# Autodesk Inventor assembly: 217-3433-Fully Constrained
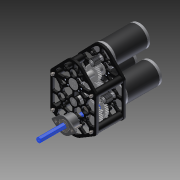
[picture p0: Inventor's stored thumbnail of the model, 180x180]
Saved by Autodesk Inventor 2014 SP1 (Build 180222100, 222)
## iProperties
Created: 2014-01-04
Part Number: 217-3433-Fully Constrained
Document SubType Name: Assembly
Designer: Moses
Mass: 6071.56 g
Surface Area: 3557.48 cm^2
Volume: 1472.05 cm^3
Density: 4.12457 g/cm^3
Title: 217-3433-STEP.STEP
Description: STEP AP214
Creation Date: 2013-12-10
Sending System: SolidWorks 2013
Preprocessor: SwSTEP 2.0
Author: Moses
## Documents named in this file (44)
- C:\Users\Arpan\Documents\GitHub\2014buildCAD\chassisdrivetrain\gearbot\217-3433 (3 CIM Gearbox - WC)\217-3433-Fully Constrained.iam
- C:\Users\Arpan\Documents\GitHub\2014buildCAD\chassisdrivetrain\gearbot\217-3433 (3 CIM Gearbox - WC)\217-2428-027 Rev1_97414A630.ipt
- C:\Users\Arpan\Documents\GitHub\2014buildCAD\chassisdrivetrain\gearbot\217-3433 (3 CIM Gearbox - WC)\217-3423-005 Rev1.ipt
- C:\Users\Arpan\Documents\GitHub\2014buildCAD\chassisdrivetrain\gearbot\217-3433 (3 CIM Gearbox - WC)\217-3195-200 Rev1.iam
- C:\Users\Arpan\Documents\GitHub\2014buildCAD\chassisdrivetrain\gearbot\217-3433 (3 CIM Gearbox - WC)\217-3489.ipt
- C:\Users\Arpan\Documents\GitHub\2014buildCAD\chassisdrivetrain\gearbot\217-3433 (3 CIM Gearbox - WC)\217-3423-006 Rev1.ipt
- C:\Users\Arpan\Documents\GitHub\2014buildCAD\chassisdrivetrain\gearbot\217-3433 (3 CIM Gearbox - WC)\217-3423-008 Rev1.ipt
- C:\Users\Arpan\Documents\GitHub\2014buildCAD\chassisdrivetrain\gearbot\217-3433 (3 CIM Gearbox - WC)\217-3423-009 Rev1.ipt
- C:\Users\Arpan\Documents\GitHub\2014buildCAD\chassisdrivetrain\gearbot\217-3433 (3 CIM Gearbox - WC)\217-2778-001 Rev2_NCQ8A075-050M.iam
- C:\Users\Arpan\Documents\GitHub\2014buildCAD\chassisdrivetrain\gearbot\217-3433 (3 CIM Gearbox - WC)\217-2731.ipt
- C:\Users\Arpan\Documents\GitHub\2014buildCAD\chassisdrivetrain\gearbot\217-3433 (3 CIM Gearbox - WC)\217-2733.ipt
- C:\Users\Arpan\Documents\GitHub\2014buildCAD\chassisdrivetrain\gearbot\217-3433 (3 CIM Gearbox - WC)\217-2734.ipt
- C:\Users\Arpan\Documents\GitHub\2014buildCAD\chassisdrivetrain\gearbot\217-3433 (3 CIM Gearbox - WC)\217-2743.ipt
- C:\Users\Arpan\Documents\GitHub\2014buildCAD\chassisdrivetrain\gearbot\217-3433 (3 CIM Gearbox - WC)\217-2614-002_98430A132.ipt
- C:\Users\Arpan\Documents\GitHub\2014buildCAD\chassisdrivetrain\gearbot\217-3433 (3 CIM Gearbox - WC)\217-3421-007 Rev1.ipt
- C:\Users\Arpan\Documents\GitHub\2014buildCAD\chassisdrivetrain\gearbot\217-3433 (3 CIM Gearbox - WC)\217-3421-009 Rev1.ipt
- C:\Users\Arpan\Documents\GitHub\2014buildCAD\chassisdrivetrain\gearbot\217-3433 (3 CIM Gearbox - WC)\217-3421-010 Rev1.ipt
- C:\Users\Arpan\Documents\GitHub\2014buildCAD\chassisdrivetrain\gearbot\217-3433 (3 CIM Gearbox - WC)\217-3421-011 Rev2_97633A200.ipt
- C:\Users\Arpan\Documents\GitHub\2014buildCAD\chassisdrivetrain\gearbot\217-3433 (3 CIM Gearbox - WC)\217-3422-007 Rev1.ipt
- C:\Users\Arpan\Documents\GitHub\2014buildCAD\chassisdrivetrain\gearbot\217-3433 (3 CIM Gearbox - WC)\217-3423-014 Rev1.ipt
- C:\Users\Arpan\Documents\GitHub\2014buildCAD\chassisdrivetrain\gearbot\217-3433 (3 CIM Gearbox - WC)\217-3423-016 Rev1.ipt
- C:\Users\Arpan\Documents\GitHub\2014buildCAD\chassisdrivetrain\gearbot\217-3433 (3 CIM Gearbox - WC)\217-3424-003 Rev1.ipt
- C:\Users\Arpan\Documents\GitHub\2014buildCAD\chassisdrivetrain\gearbot\217-3433 (3 CIM Gearbox - WC)\217-2761-001 rev1.ipt
- C:\Users\Arpan\Documents\GitHub\2014buildCAD\chassisdrivetrain\gearbot\217-3433 (3 CIM Gearbox - WC)\217-3210-001 Rev1_30t.ipt
- C:\Users\Arpan\Documents\GitHub\2014buildCAD\chassisdrivetrain\gearbot\217-3433 (3 CIM Gearbox - WC)\217-3215-001 Rev1_42t.ipt
- C:\Users\Arpan\Documents\GitHub\2014buildCAD\chassisdrivetrain\gearbot\217-3433 (3 CIM Gearbox - WC)\217-3414-001 Rev1_14t Steel Pinion.ipt
- C:\Users\Arpan\Documents\GitHub\2014buildCAD\chassisdrivetrain\gearbot\217-3433 (3 CIM Gearbox - WC)\217-3418-001 Rev2_44t.ipt
- C:\Users\Arpan\Documents\GitHub\2014buildCAD\chassisdrivetrain\gearbot\217-3433 (3 CIM Gearbox - WC)\217-3420-001 Rev2_60t.ipt
- C:\Users\Arpan\Documents\GitHub\2014buildCAD\chassisdrivetrain\gearbot\217-3433 (3 CIM Gearbox - WC)\217-3100-001_14t.ipt
- C:\Users\Arpan\Documents\GitHub\2014buildCAD\chassisdrivetrain\gearbot\217-3433 (3 CIM Gearbox - WC)\217-2705-001_30t.ipt
- C:\Users\Arpan\Documents\GitHub\2014buildCAD\chassisdrivetrain\gearbot\217-3433 (3 CIM Gearbox - WC)\217-2000.ipt
- C:\Users\Arpan\Documents\GitHub\2014buildCAD\chassisdrivetrain\gearbot\217-3433 (3 CIM Gearbox - WC)\217-3433-001 Rev1_Default_As Machined_.ipt
- C:\Users\Arpan\Documents\GitHub\2014buildCAD\chassisdrivetrain\gearbot\217-3433 (3 CIM Gearbox - WC)\217-3423-003 Rev1.ipt
- C:\Users\Arpan\Documents\GitHub\2014buildCAD\chassisdrivetrain\gearbot\217-3433 (3 CIM Gearbox - WC)\217-3424-005 Rev1.ipt
- C:\Users\Arpan\Documents\GitHub\2014buildCAD\chassisdrivetrain\gearbot\217-3433 (3 CIM Gearbox - WC)\217-3433-003 Rev1.ipt
- C:\Users\Arpan\Documents\GitHub\2014buildCAD\chassisdrivetrain\gearbot\217-3433 (3 CIM Gearbox - WC)\217-3256-001 Rev1.ipt
- C:\Users\Arpan\Documents\GitHub\2014buildCAD\chassisdrivetrain\gearbot\217-3433 (3 CIM Gearbox - WC)\217-3261-001 Rev1.ipt
- C:\Users\Arpan\Documents\GitHub\2014buildCAD\chassisdrivetrain\gearbot\217-3433 (3 CIM Gearbox - WC)\217-3423-004 Rev1.ipt
- C:\Users\Arpan\Documents\GitHub\2014buildCAD\chassisdrivetrain\gearbot\217-3433 (3 CIM Gearbox - WC)\217-3424-002 Rev1.ipt
- C:\Users\Arpan\Documents\GitHub\2014buildCAD\chassisdrivetrain\gearbot\217-3433 (3 CIM Gearbox - WC)\217-3422-004 Rev2.ipt
- C:\Users\Arpan\Documents\GitHub\2014buildCAD\chassisdrivetrain\gearbot\217-3433 (3 CIM Gearbox - WC)\217-3257-001 Rev1.ipt
- C:\Users\Arpan\Documents\GitHub\2014buildCAD\chassisdrivetrain\gearbot\217-3433 (3 CIM Gearbox - WC)\217-3263-001 Rev1.ipt
- C:\Users\Arpan\Documents\GitHub\2014buildCAD\chassisdrivetrain\gearbot\217-3433 (3 CIM Gearbox - WC)\217-3259-001 Rev1.ipt
- C:\Users\Arpan\Documents\GitHub\2014buildCAD\chassisdrivetrain\gearbot\217-3433 (3 CIM Gearbox - WC)\217-2758-001 Rev1.ipt
## Components (78 placed, 78 different names)
1. 217-2428-027 Rev1_97414A630_1 — Insert:47, Mate:62, Rotation:10
2. 217-3423-005 Rev1_2 — Insert:32, Insert:33, Insert:34, Insert:35, Insert:36, Mate:61
3. 217-3195-200 Rev1_3 [sub-assembly] — Flush:4, Mate:60, Mate:61, Rotation:9, Angle:13
4. 217-3489_4 — Insert:47, Mate:64
5. 217-3423-006 Rev1_5 — Insert:31, Insert:32
6. 217-3423-006 Rev1_6 — Insert:30, Insert:33
7. 217-3423-008 Rev1_7 — Mate:29, Mate:42, Flush:4, Mate:60, Mate:62, Mate:64
8. 217-3423-009 Rev1_8 — Mate:34, Insert:28, Rotation:2
9. 217-2778-001 Rev2_NCQ8A075-050M_9 [sub-assembly] — Insert:36, Angle:6, Angle:13
10. 217-2731_10 — Insert:22, Mate:24, Mate:29, Mate:43, Mate:45
11. 217-2733_11 — Insert:40, Insert:45
12. 217-2733_12 — Insert:15, Insert:38
13. 217-2734_13 — Insert:13, Angle:1, Flush:3, Insert:48
14. 217-2734_14 — Insert:27, Angle:2, Mate:35, Mate:36
15. 217-2743_15 — Mate:39, Mate:40
16. 217-2731_16 — Insert:12, Insert:37
17. 217-2731_17 — Insert:41, Insert:46
18. 217-2614-002_98430A132_18 — Mate:27, Mate:47, Rotation:13
19. 217-2614-002_98430A132_19 — Mate:28, Mate:48, Rotation:16
20. 217-2614-002_98430A132_20 — Mate:51, Mate:54, Rotation:12
21. 217-2614-002_98430A132_21 — Mate:52, Mate:53, Rotation:15
22. 217-2614-002_98430A132_22 — Mate:25, Mate:50, Rotation:11
23. 217-2614-002_98430A132_23 — Mate:26, Mate:49, Rotation:14
24. 217-3421-007 Rev1_24 — Insert:34
25. 217-3421-007 Rev1_25 — Insert:35
26. 217-3421-009 Rev1_26 — Insert:19
27. 217-3421-009 Rev1_27 — Insert:17
28. 217-3421-009 Rev1_28 — Insert:18
29. 217-3421-009 Rev1_29 — Insert:21
30. 217-3421-009 Rev1_30 — Insert:20
31. 217-3421-009 Rev1_31 — Insert:16
32. 217-3421-010 Rev1_32 — Insert:26
33. 217-3421-010 Rev1_33 — Insert:25
34. 217-3421-010 Rev1_34 — Insert:23
35. 217-3421-010 Rev1_35 — Insert:24
36. 217-3421-011 Rev2_97633A200_36 — Insert:29, Rotation:4
37. 217-3422-007 Rev1_37 — Flush:1, Mate:5, Mate:7
38. 217-3422-007 Rev1_38 — Flush:2, Mate:6, Mate:8
39. 217-3423-014 Rev1_39 — Insert:28, Mate:42
40. 217-3423-016 Rev1_40 — Mate:45, Mate:46
41. 217-3423-016 Rev1_41 — Mate:43, Mate:44
42. 217-3423-016 Rev1_42 — Mate:23, Mate:24
43. 217-3424-003 Rev1_43 — Insert:59
44. 217-3424-003 Rev1_44 — Insert:60
45. 217-3424-003 Rev1_45 — Insert:58
46. 217-3424-003 Rev1_46 — Insert:57
47. 217-2761-001 rev1_47 — Mate:20, Mate:21, Mate:22
48. 217-2761-001 rev1_48 — Mate:4, Mate:13, Mate:14
49. 217-2761-001 rev1_49 — Mate:15, Mate:16, Mate:18
50. 217-3210-001 Rev1_30t_50 — Insert:44, Angle:11, Insert:45, Rotation:18
51. 217-3215-001 Rev1_42t_51 — Insert:43, Mate:59, Angle:10, Insert:44, Rotation:6, Rotation:7, Rotation:8
52. 217-3414-001 Rev1_14t Steel Pinion_52 — Mate:3, Mate:11, Mate:52, Mate:54, Rotation:7, Rotation:12, Rotation:15
53. 217-3414-001 Rev1_14t Steel Pinion_53 — Mate:2, Mate:10, Mate:47, Mate:48, Rotation:8, Rotation:13, Rotation:16
54. 217-3414-001 Rev1_14t Steel Pinion_54 — Mate:1, Mate:9, Mate:49, Mate:50, Rotation:5, Rotation:11, Rotation:14
55. 217-3418-001 Rev2_44t_55 — Mate:37, Fast Rotation Ratio:3, Mate:40, Mate:41, Rotation:18
56. 217-3420-001 Rev2_60t_56 — Insert:27, Slow Rotation Ratio:1, Mate:41, Rotation:17
57. 217-3100-001_14t_57 — Angle:7, Insert:39, Rotation:17
58. 217-2705-001_30t_58 — Angle:8, Insert:42, Rotation:5, Rotation:6
59. 217-2000_59 — Insert:2, Mate:2, Mate:10, Mate:19, Mate:20, Mate:21, Mate:22, Mate:27, Mate:28
60. 217-2000_60 — Insert:3, Mate:3, Mate:4, Mate:11, Mate:12, Mate:13, Mate:14, Mate:51, Mate:53
61. 217-2000_61 — Insert:1, Mate:1, Mate:9, Mate:15, Mate:16, Mate:17, Mate:18, Mate:25, Mate:26
62. 217-3433-001 Rev1_Default<As Machined>_62 — Insert:1, Insert:2, Insert:3, Insert:4, Insert:7, Insert:8, Insert:11, Insert:16, Insert:17, Insert:18, Insert:19, Insert:20, Insert:21, Mate:12, Mate:17, Mate:19, Insert:22, Mate:23, Insert:23, Insert:24, Insert:25, Insert:26, Insert:30, Insert:31, Angle:6, Mate:44, Mate:46, Insert:40, Insert:41
63. 217-3433-001 Rev1_Default<As Machined>_63 — Insert:5, Insert:6, Insert:9, Insert:10, Insert:12, Mate:5, Mate:6, Insert:14, Insert:15, Mate:30, Mate:31, Mate:32, Mate:33, Mate:34, Mate:35, Mate:37, Mate:38, Mate:39, Insert:58, Insert:57, Insert:60, Insert:59
64. 217-3423-003 Rev1_64 — Angle:1, Slow Rotation Ratio:1, Angle:2, Rotation:2, Mate:36, Fast Rotation Ratio:3, Mate:38, Flush:3, Angle:3, Angle:4, Angle:5, Insert:29, Rotation:4, Rotation:9, Rotation:10
65. 217-3424-005 Rev1_65 — Insert:38, Angle:7, Insert:39, Angle:9, Mate:59, Angle:10, Angle:11
66. 217-3433-003 Rev1_66 — Insert:37, Angle:8, Insert:42, Angle:12
67. 217-3256-001 Rev1_67 — Insert:43, Angle:9
68. 217-3261-001 Rev1_68 — Insert:46, Angle:12
69. 217-3423-004 Rev1_69
70. 217-3424-002 Rev1_70 — Insert:6, Insert:7
71. 217-3424-002 Rev1_71 — Insert:10, Insert:11
72. 217-3424-002 Rev1_72 — Insert:4, Insert:5
73. 217-3424-002 Rev1_73 — Insert:8, Insert:9
74. 217-3422-004 Rev2_74 — Insert:13, Flush:1, Flush:2, Mate:7, Mate:8, Insert:14
75. 217-3257-001 Rev1_75 — Mate:33, Angle:3
76. 217-3263-001 Rev1_76 — Mate:30, Insert:48, Insert:49
77. 217-3259-001 Rev1_77 — Mate:31, Angle:5, Mate:63, Insert:49
78. 217-2758-001 Rev1_78 — Mate:32, Angle:4, Mate:63
## Relationships (148: Mate 60, Insert 53, RelateRotation 18, Angle 13, Flush 4)
- Insert:1: 217-2000_61 ↔ 217-3433-001 Rev1_Default<As Machined>_62
- Insert:2: 217-2000_59 ↔ 217-3433-001 Rev1_Default<As Machined>_62
- Insert:3: 217-2000_60 ↔ 217-3433-001 Rev1_Default<As Machined>_62
- Mate:1 (10.2113 mm): 217-3414-001 Rev1_14t Steel Pinion_54 ↔ 217-2000_61
- Mate:2 (10.2113 mm): 217-3414-001 Rev1_14t Steel Pinion_53 ↔ 217-2000_59
- Mate:3 (10.2113 mm): 217-3414-001 Rev1_14t Steel Pinion_52 ↔ 217-2000_60
- Mate:4: 217-2761-001 rev1_48 ↔ 217-2000_60
- Insert:4: 217-3433-001 Rev1_Default<As Machined>_62 ↔ 217-3424-002 Rev1_72
- Insert:5: 217-3433-001 Rev1_Default<As Machined>_63 ↔ 217-3424-002 Rev1_72
- Insert:6: 217-3433-001 Rev1_Default<As Machined>_63 ↔ 217-3424-002 Rev1_70
- Insert:7: 217-3433-001 Rev1_Default<As Machined>_62 ↔ 217-3424-002 Rev1_70
- Insert:8: 217-3433-001 Rev1_Default<As Machined>_62 ↔ 217-3424-002 Rev1_73
- Insert:9: 217-3433-001 Rev1_Default<As Machined>_63 ↔ 217-3424-002 Rev1_73
- Insert:10: 217-3433-001 Rev1_Default<As Machined>_63 ↔ 217-3424-002 Rev1_71
- Insert:11: 217-3433-001 Rev1_Default<As Machined>_62 ↔ 217-3424-002 Rev1_71
- Insert:12: 217-2731_16 ↔ 217-3433-001 Rev1_Default<As Machined>_63
- Insert:13: 217-2734_13 ↔ 217-3422-004 Rev2_74
- Flush:1: 217-3422-007 Rev1_37 ↔ 217-3422-004 Rev2_74
- Flush:2: 217-3422-007 Rev1_38 ↔ 217-3422-004 Rev2_74
- Mate:5: 217-3422-007 Rev1_37 ↔ 217-3433-001 Rev1_Default<As Machined>_63
- Mate:6: 217-3422-007 Rev1_38 ↔ 217-3433-001 Rev1_Default<As Machined>_63
- Mate:7: 217-3422-007 Rev1_37 ↔ 217-3422-004 Rev2_74
- Mate:8: 217-3422-007 Rev1_38 ↔ 217-3422-004 Rev2_74
- Insert:14: 217-3433-001 Rev1_Default<As Machined>_63 ↔ 217-3422-004 Rev2_74
- Insert:15: 217-2733_12 ↔ 217-3433-001 Rev1_Default<As Machined>_63
- Insert:16: 217-3421-009 Rev1_31 ↔ 217-3433-001 Rev1_Default<As Machined>_62
- Insert:17: 217-3421-009 Rev1_27 ↔ 217-3433-001 Rev1_Default<As Machined>_62
- Insert:18: 217-3421-009 Rev1_28 ↔ 217-3433-001 Rev1_Default<As Machined>_62
- Insert:19: 217-3421-009 Rev1_26 ↔ 217-3433-001 Rev1_Default<As Machined>_62
- Mate:9: 217-3414-001 Rev1_14t Steel Pinion_54 ↔ 217-2000_61
- Mate:10: 217-3414-001 Rev1_14t Steel Pinion_53 ↔ 217-2000_59
- Mate:11: 217-3414-001 Rev1_14t Steel Pinion_52 ↔ 217-2000_60
- Insert:20: 217-3421-009 Rev1_30 ↔ 217-3433-001 Rev1_Default<As Machined>_62
- Insert:21: 217-3421-009 Rev1_29 ↔ 217-3433-001 Rev1_Default<As Machined>_62
- Mate:12: 217-2000_60 ↔ 217-3433-001 Rev1_Default<As Machined>_62
- Mate:13: 217-2761-001 rev1_48 ↔ 217-2000_60
- Mate:14: 217-2761-001 rev1_48 ↔ 217-2000_60
- Mate:15: 217-2761-001 rev1_49 ↔ 217-2000_61
- Mate:16: 217-2761-001 rev1_49 ↔ 217-2000_61
- Mate:17: 217-2000_61 ↔ 217-3433-001 Rev1_Default<As Machined>_62
- Mate:18: 217-2761-001 rev1_49 ↔ 217-2000_61
- Mate:19: 217-2000_59 ↔ 217-3433-001 Rev1_Default<As Machined>_62
- Mate:20: 217-2761-001 rev1_47 ↔ 217-2000_59
- Mate:21: 217-2761-001 rev1_47 ↔ 217-2000_59
- Mate:22: 217-2761-001 rev1_47 ↔ 217-2000_59
- Insert:22: 217-2731_10 ↔ 217-3433-001 Rev1_Default<As Machined>_62
- Mate:23: 217-3423-016 Rev1_42 ↔ 217-3433-001 Rev1_Default<As Machined>_62
- Mate:24: 217-2731_10 ↔ 217-3423-016 Rev1_42
- Mate:25: 217-2614-002_98430A132_22 ↔ 217-2000_61
- Mate:26: 217-2614-002_98430A132_23 ↔ 217-2000_61
- Mate:27: 217-2614-002_98430A132_18 ↔ 217-2000_59
- Mate:28: 217-2614-002_98430A132_19 ↔ 217-2000_59
- Mate:29: 217-3423-008 Rev1_7 ↔ 217-2731_10
- Angle:1 (0 deg): 217-2734_13 ↔ 217-3423-003 Rev1_64
- Insert:23: 217-3421-010 Rev1_34 ↔ 217-3433-001 Rev1_Default<As Machined>_62
- Insert:24: 217-3421-010 Rev1_35 ↔ 217-3433-001 Rev1_Default<As Machined>_62
- Insert:25: 217-3421-010 Rev1_33 ↔ 217-3433-001 Rev1_Default<As Machined>_62
- Insert:26: 217-3421-010 Rev1_32 ↔ 217-3433-001 Rev1_Default<As Machined>_62
- Mate:30: 217-3433-001 Rev1_Default<As Machined>_63 ↔ 217-3263-001 Rev1_76
- Mate:31: 217-3433-001 Rev1_Default<As Machined>_63 ↔ 217-3259-001 Rev1_77
- Mate:32: 217-3433-001 Rev1_Default<As Machined>_63 ↔ 217-2758-001 Rev1_78
- Mate:33: 217-3433-001 Rev1_Default<As Machined>_63 ↔ 217-3257-001 Rev1_75
- Insert:27: 217-2734_14 ↔ 217-3420-001 Rev2_60t_56
- Mate:34: 217-3423-009 Rev1_8 ↔ 217-3433-001 Rev1_Default<As Machined>_63
- Insert:28: 217-3423-009 Rev1_8 ↔ 217-3423-014 Rev1_39
- Slow Rotation Ratio:1 [RelateRotation] (1 ul): 217-3420-001 Rev2_60t_56 ↔ 217-3423-003 Rev1_64
- Angle:2 (0 deg): 217-2734_14 ↔ 217-3423-003 Rev1_64
- Rotation:2 [RelateRotation] (1 ul): 217-3423-009 Rev1_8 ↔ 217-3423-003 Rev1_64
- Mate:35: 217-2734_14 ↔ 217-3433-001 Rev1_Default<As Machined>_63
- Mate:36: 217-2734_14 ↔ 217-3423-003 Rev1_64
- Mate:37: 217-3418-001 Rev2_44t_55 ↔ 217-3433-001 Rev1_Default<As Machined>_63
- Fast Rotation Ratio:3 [RelateRotation] (1 ul): 217-3418-001 Rev2_44t_55 ↔ 217-3423-003 Rev1_64
- Mate:38: 217-3433-001 Rev1_Default<As Machined>_63 ↔ 217-3423-003 Rev1_64
- Flush:3 (74.8347 mm): 217-2734_13 ↔ 217-3423-003 Rev1_64
- Angle:3 (0 deg): 217-3423-003 Rev1_64 ↔ 217-3257-001 Rev1_75
- Angle:4 (0 deg): 217-3423-003 Rev1_64 ↔ 217-2758-001 Rev1_78
- Angle:5 (0 deg): 217-3423-003 Rev1_64 ↔ 217-3259-001 Rev1_77
- Mate:39: 217-2743_15 ↔ 217-3433-001 Rev1_Default<As Machined>_63
- Mate:40: 217-2743_15 ↔ 217-3418-001 Rev2_44t_55
- Mate:41 (18.1613 mm): 217-3418-001 Rev2_44t_55 ↔ 217-3420-001 Rev2_60t_56
- Mate:42: 217-3423-008 Rev1_7 ↔ 217-3423-014 Rev1_39
- Insert:29: 217-3421-011 Rev2_97633A200_36 ↔ 217-3423-003 Rev1_64
- Rotation:4 [RelateRotation] (1 ul): 217-3421-011 Rev2_97633A200_36 ↔ 217-3423-003 Rev1_64
- Insert:30: 217-3423-006 Rev1_6 ↔ 217-3433-001 Rev1_Default<As Machined>_62
- Insert:31: 217-3423-006 Rev1_5 ↔ 217-3433-001 Rev1_Default<As Machined>_62
- Insert:32: 217-3423-005 Rev1_2 ↔ 217-3423-006 Rev1_5
- Insert:33: 217-3423-005 Rev1_2 ↔ 217-3423-006 Rev1_6
- Insert:34: 217-3423-005 Rev1_2 ↔ 217-3421-007 Rev1_24
- Insert:35: 217-3423-005 Rev1_2 ↔ 217-3421-007 Rev1_25
- Flush:4: 217-3195-200 Rev1_3 ↔ 217-3423-008 Rev1_7
- Insert:36: 217-3423-005 Rev1_2 ↔ 217-2778-001 Rev2_NCQ8A075-050M_9
- Angle:6 (0 deg): 217-2778-001 Rev2_NCQ8A075-050M_9 ↔ 217-3433-001 Rev1_Default<As Machined>_62
- Mate:43: 217-2731_10 ↔ 217-3423-016 Rev1_41
- Mate:44: 217-3423-016 Rev1_41 ↔ 217-3433-001 Rev1_Default<As Machined>_62
- Mate:45: 217-2731_10 ↔ 217-3423-016 Rev1_40
- Mate:46: 217-3423-016 Rev1_40 ↔ 217-3433-001 Rev1_Default<As Machined>_62
- Insert:37: 217-2731_16 ↔ 217-3433-003 Rev1_66
- Insert:38: 217-2733_12 ↔ 217-3424-005 Rev1_65
- Mate:47: 217-2614-002_98430A132_18 ↔ 217-3414-001 Rev1_14t Steel Pinion_53
- Mate:48: 217-2614-002_98430A132_19 ↔ 217-3414-001 Rev1_14t Steel Pinion_53
- Mate:49: 217-2614-002_98430A132_23 ↔ 217-3414-001 Rev1_14t Steel Pinion_54
- Mate:50: 217-2614-002_98430A132_22 ↔ 217-3414-001 Rev1_14t Steel Pinion_54
- Mate:51: 217-2614-002_98430A132_20 ↔ 217-2000_60
- Mate:52: 217-2614-002_98430A132_21 ↔ 217-3414-001 Rev1_14t Steel Pinion_52
- Mate:53: 217-2614-002_98430A132_21 ↔ 217-2000_60
- Mate:54: 217-2614-002_98430A132_20 ↔ 217-3414-001 Rev1_14t Steel Pinion_52
- Insert:58 (3.175 mm): 217-3424-003 Rev1_45 ↔ 217-3433-001 Rev1_Default<As Machined>_63
- Insert:57 (3.175 mm): 217-3424-003 Rev1_46 ↔ 217-3433-001 Rev1_Default<As Machined>_63
- Insert:60 (3.175 mm): 217-3424-003 Rev1_44 ↔ 217-3433-001 Rev1_Default<As Machined>_63
- Insert:59 (3.175 mm): 217-3424-003 Rev1_43 ↔ 217-3433-001 Rev1_Default<As Machined>_63
- Angle:7 (0 deg): 217-3100-001_14t_57 ↔ 217-3424-005 Rev1_65
- Insert:39: 217-3100-001_14t_57 ↔ 217-3424-005 Rev1_65
- Insert:40: 217-2733_11 ↔ 217-3433-001 Rev1_Default<As Machined>_62
- Insert:41: 217-2731_17 ↔ 217-3433-001 Rev1_Default<As Machined>_62
- Angle:8 (0 deg): 217-2705-001_30t_58 ↔ 217-3433-003 Rev1_66
- Insert:42: 217-2705-001_30t_58 ↔ 217-3433-003 Rev1_66
- Insert:43: 217-3215-001 Rev1_42t_51 ↔ 217-3256-001 Rev1_67
- Angle:9 (0 deg): 217-3424-005 Rev1_65 ↔ 217-3256-001 Rev1_67
- Mate:59: 217-3215-001 Rev1_42t_51 ↔ 217-3424-005 Rev1_65
- Angle:10 (0 deg): 217-3215-001 Rev1_42t_51 ↔ 217-3424-005 Rev1_65
- Insert:44: 217-3210-001 Rev1_30t_50 ↔ 217-3215-001 Rev1_42t_51
- Angle:11 (0 deg): 217-3210-001 Rev1_30t_50 ↔ 217-3424-005 Rev1_65
- Insert:45: 217-2733_11 ↔ 217-3210-001 Rev1_30t_50
- Insert:46: 217-2731_17 ↔ 217-3261-001 Rev1_68
- Angle:12 (0 deg): 217-3433-003 Rev1_66 ↔ 217-3261-001 Rev1_68
- Rotation:5 [RelateRotation] (2.1429 ul): 217-3414-001 Rev1_14t Steel Pinion_54 ↔ 217-2705-001_30t_58
- Rotation:6 [RelateRotation] (0.7143 ul): 217-3215-001 Rev1_42t_51 ↔ 217-2705-001_30t_58
- Rotation:7 [RelateRotation] (3 ul): 217-3215-001 Rev1_42t_51 ↔ 217-3414-001 Rev1_14t Steel Pinion_52
- Rotation:8 [RelateRotation] (3 ul): 217-3215-001 Rev1_42t_51 ↔ 217-3414-001 Rev1_14t Steel Pinion_53
- Mate:60: 217-3195-200 Rev1_3 ↔ 217-3423-008 Rev1_7
- Mate:61 (4.7711 mm): 217-3423-005 Rev1_2 ↔ 217-3195-200 Rev1_3
- Rotation:9 [RelateRotation] (1 ul): 217-3195-200 Rev1_3 ↔ 217-3423-003 Rev1_64
- Insert:47: 217-2428-027 Rev1_97414A630_1 ↔ 217-3489_4
- Mate:62 (0.0908 mm): 217-2428-027 Rev1_97414A630_1 ↔ 217-3423-008 Rev1_7
- Angle:13 (0 deg): 217-3195-200 Rev1_3 ↔ 217-2778-001 Rev2_NCQ8A075-050M_9
- Mate:63 (2.3303 mm): 217-3259-001 Rev1_77 ↔ 217-2758-001 Rev1_78
- Insert:48: 217-2734_13 ↔ 217-3263-001 Rev1_76
- Insert:49: 217-3263-001 Rev1_76 ↔ 217-3259-001 Rev1_77
- Mate:64: 217-3489_4 ↔ 217-3423-008 Rev1_7
- Rotation:10 [RelateRotation] (1 ul): 217-2428-027 Rev1_97414A630_1 ↔ 217-3423-003 Rev1_64
- Rotation:11 [RelateRotation] (1 ul): 217-2614-002_98430A132_22 ↔ 217-3414-001 Rev1_14t Steel Pinion_54
- Rotation:12 [RelateRotation] (1 ul): 217-2614-002_98430A132_20 ↔ 217-3414-001 Rev1_14t Steel Pinion_52
- Rotation:13 [RelateRotation] (1 ul): 217-2614-002_98430A132_18 ↔ 217-3414-001 Rev1_14t Steel Pinion_53
- Rotation:14 [RelateRotation] (1 ul): 217-2614-002_98430A132_23 ↔ 217-3414-001 Rev1_14t Steel Pinion_54
- Rotation:15 [RelateRotation] (1 ul): 217-2614-002_98430A132_21 ↔ 217-3414-001 Rev1_14t Steel Pinion_52
- Rotation:16 [RelateRotation] (1 ul): 217-2614-002_98430A132_19 ↔ 217-3414-001 Rev1_14t Steel Pinion_53
- Rotation:17 [RelateRotation] (0.2333 ul): 217-3420-001 Rev2_60t_56 ↔ 217-3100-001_14t_57
- Rotation:18 [RelateRotation] (0.6818 ul): 217-3210-001 Rev1_30t_50 ↔ 217-3418-001 Rev2_44t_55
